# Autodesk Inventor assembly: Extender
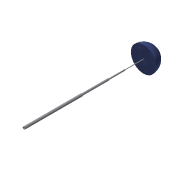
[picture p0: Inventor's stored thumbnail of the model, 180x180]
Saved by Autodesk Inventor 2015 (Build 190159000, 159)
## iProperties
Created: 2015-01-31
Part Number: Extender
Document SubType Name: Assembly
Designer: Tanner
Author: Tanner
## Documents named in this file (6)
- C:\Users\Tanner\Documents\GitHub\FIRST-Team-1719-CAD-Team\2015 Robot CAD\Devices\Extender\Extender.iam
- C:\Users\Tanner\Documents\GitHub\FIRST-Team-1719-CAD-Team\2015 Robot CAD\Devices\Extender\Tubing\Extender - .5 in tube.ipt
- C:\Users\Tanner\Documents\GitHub\FIRST-Team-1719-CAD-Team\2015 Robot CAD\Devices\Extender\Tubing\Extender - .25 tube.ipt
- C:\Users\Tanner\Documents\GitHub\FIRST-Team-1719-CAD-Team\2015 Robot CAD\Devices\Extender\Tubing\Extender - .75 in tube.ipt
- C:\Users\Tanner\Documents\GitHub\FIRST-Team-1719-CAD-Team\2015 Robot CAD\Devices\Extender\Tubing\Extender - 1 in tube.ipt
- C:\Users\Tanner\Documents\GitHub\FIRST-Team-1719-CAD-Team\2015 Robot CAD\Devices\Extender\Misc\Umbrella.ipt
## Components (5 placed, 5 different names)
1. Extender - .5 in tube:1 — Mate:2, Mate:3
2. Extender - .25 tube:1 — Mate:3, Insert:1
3. Extender - .75 in tube:1 — Mate:1, Mate:2
4. Extender - 1 in tube:1 — Mate:1
5. Umbrella:1 — Insert:1
## Relationships (4: Mate 3, Insert 1)
- Mate:1: Extender - .75 in tube:1 ↔ Extender - 1 in tube:1
- Mate:2: Extender - .5 in tube:1 ↔ Extender - .75 in tube:1
- Mate:3: Extender - .5 in tube:1 ↔ Extender - .25 tube:1
- Insert:1: Extender - .25 tube:1 ↔ Umbrella:1
